# Autodesk Inventor assembly: Computer box with equipment
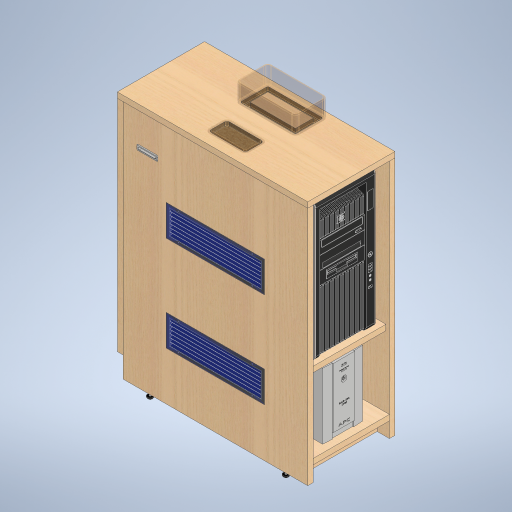
[picture p0: Inventor's stored thumbnail of the model, 512x512]
Saved by Autodesk Inventor 2024 (Build 280153000, 153)
## iProperties
Created: 2021-12-30
Part Number: Computer box with equipment
Document SubType Name: Assembly
Designer: sauliusd
Author: sauliusd
## Documents named in this file (3)
- C:\W4INV 2024 Design\PROJECTS\Samples\Macro DEMO\7 Computer Box\Computer box with equipment.iam
- C:\W4INV 2024 Design\PROJECTS\Samples\Macro DEMO\7 Computer Box\Computer box.iam
- C:\W4INV 2024 Design\PROJECTS\Samples\Macro DEMO\7 Computer Box\Computer equipment.iam
## Components (2 placed, 2 different names)
1. Computer box:1 [sub-assembly]
2. Computer equipment:1 [sub-assembly] — Flush:1, Flush:2, Flush:3
## Relationships (3: Flush 3)
- Flush:1: Computer equipment:1
- Flush:2: Computer equipment:1
- Flush:3: Computer equipment:1
